# Autodesk Inventor assembly: Assembly10(Suction houe sub assembly)
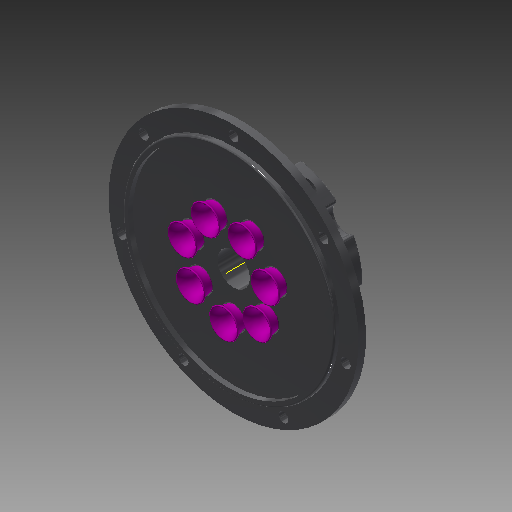
[picture p0: Inventor's stored thumbnail of the model, 512x512]
Saved by Autodesk Inventor 2018 (Build 220112000, 112)
## iProperties
Created: 2023-05-02
Part Number: Assembly10(Suction houe sub assembly)
Document SubType Name: Assembly
Designer: Habib Mohamed
Author: Habib Mohamed
## Documents named in this file (3)
- D:\Inventor\My projects\Rotary Engine\Assembly\Assembly10(Suction houe sub assembly).iam
- D:\Inventor\My projects\Rotary Engine\Block 2 (Suction Housing).ipt
- D:\Inventor\My projects\Rotary Engine\Component 1(Venturi).ipt
## Components (8 placed, 2 different names)
1. Block 2 (Suction Housing):1 — Mate:1, Mate:2, Mate:3
2. Component 1(Venturi):1 — Mate:1, Mate:2
3. Component 1(Venturi):2
4. Component 1(Venturi):3
5. Component 1(Venturi):4
6. Component 1(Venturi):5
7. Component 1(Venturi):6
8. Component 1(Venturi):7
## Component patterns: (7 elements, first: Component 1(Venturi):1)
## Relationships (3: Mate 3)
- Mate:1: Block 2 (Suction Housing):1 ↔ Component 1(Venturi):1
- Mate:2: Block 2 (Suction Housing):1 ↔ Component 1(Venturi):1
- Mate:3: Block 2 (Suction Housing):1
